# Autodesk Inventor assembly: 95654
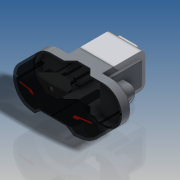
[picture p0: Inventor's stored thumbnail of the model, 180x180]
Saved by Autodesk Inventor 2016 SP2 (Build 200236200, 236)
## iProperties
Created: 2015-08-24
Part Number: 95654
Document SubType Name: Assembly
Designer: D. Kohfeld
Mass: 15.1454 g
Surface Area: 213.312 cm^2
Volume: 13.746 cm^3
Density: 1.1018 g/cm^3
Author: D. Kohfeld
## Documents named in this file (8)
- A:\LEGO Pieces\EV3\95654.iam
- A:\LEGO Pieces\EV3\99378-LtBluishGray.ipt
- A:\LEGO Pieces\EV3\99393-LtBluishGray.ipt
- A:\LEGO Pieces\EV3\11016-Black.ipt
- A:\LEGO Pieces\EV3\99376-White.ipt
- A:\LEGO Pieces\EV3\99392p01-TransBlackIRLens.ipt
- A:\LEGO Pieces\EV3\54732b-LtBluishGray.ipt
- A:\LEGO Pieces\EV3\99961-TransClear.ipt
## Components (8 placed, 7 different names)
1. 99378-LtBluishGray:1 — Flush:1, Mate:1, Mate:5, Angle:1, Mate:6, Mate:7, Angle:2, Mate:8, Flush:3, Flush:4, Mate:9, Flush:5, Flush:6
2. 99393-LtBluishGray:1 — Mate:5, Angle:1, Mate:6
3. 99393-LtBluishGray:2 — Mate:7, Angle:2, Mate:8
4. 11016-Black:1 — Flush:6, Mate:10, Mate:11, Mate:12, Tangent:1, Angle:3
5. 99376-White:1 — Flush:1, Mate:1, Mate:3, Mate:4, Flush:2, Flush:3
6. 99392p01-TransBlackIRLens:1 — Flush:4, Mate:9, Flush:5, Mate:10, Mate:11
7. 54732b-LtBluishGray:1 — Mate:3, Mate:4, Flush:2
8. 99961-TransClear:1 — Mate:12, Tangent:1, Angle:3
## Relationships (21: Mate 11, Flush 6, Angle 3, Tangent 1)
- Flush:1: 99378-LtBluishGray:1 ↔ 99376-White:1
- Mate:1: 99378-LtBluishGray:1 ↔ 99376-White:1
- Mate:3: 99376-White:1 ↔ 54732b-LtBluishGray:1
- Mate:4: 99376-White:1 ↔ 54732b-LtBluishGray:1
- Flush:2: 99376-White:1 ↔ 54732b-LtBluishGray:1
- Mate:5: 99378-LtBluishGray:1 ↔ 99393-LtBluishGray:1
- Angle:1 (0 deg): 99378-LtBluishGray:1 ↔ 99393-LtBluishGray:1
- Mate:6: 99378-LtBluishGray:1 ↔ 99393-LtBluishGray:1
- Mate:7: 99378-LtBluishGray:1 ↔ 99393-LtBluishGray:2
- Angle:2 (0 deg): 99378-LtBluishGray:1 ↔ 99393-LtBluishGray:2
- Mate:8: 99378-LtBluishGray:1 ↔ 99393-LtBluishGray:2
- Flush:3: 99378-LtBluishGray:1 ↔ 99376-White:1
- Flush:4: 99378-LtBluishGray:1 ↔ 99392p01-TransBlackIRLens:1
- Mate:9: 99378-LtBluishGray:1 ↔ 99392p01-TransBlackIRLens:1
- Flush:5: 99378-LtBluishGray:1 ↔ 99392p01-TransBlackIRLens:1
- Flush:6: 99378-LtBluishGray:1 ↔ 11016-Black:1
- Mate:10: 11016-Black:1 ↔ 99392p01-TransBlackIRLens:1
- Mate:11: 11016-Black:1 ↔ 99392p01-TransBlackIRLens:1
- Mate:12: 11016-Black:1 ↔ 99961-TransClear:1
- Tangent:1: 11016-Black:1 ↔ 99961-TransClear:1
- Angle:3 (0 deg): 11016-Black:1 ↔ 99961-TransClear:1
